# Autodesk Inventor assembly: prototype_5_batteryWithSlider
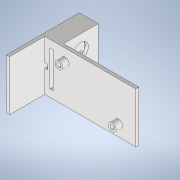
[picture p0: Inventor's stored thumbnail of the model, 180x180]
Saved by Autodesk Inventor 2022 (Build 260153000, 153)
## iProperties
Created: 2022-06-08
Part Number: prototype_5_batteryWithSlider
Document SubType Name: Assembly
Designer: tecware
Author: tecware
## Documents named in this file (3)
- C:\Users\tecware\Documents\git\calibrationKit\calibrationKit_v2\wand\prototype\New folder\prototype_6_batteryWithSlider.iam
- C:\Users\tecware\Documents\git\calibrationKit\calibrationKit_v2\wand\prototype\New folder\prototype_6_batteryPart.ipt
- C:\Users\tecware\Documents\git\calibrationKit\calibrationKit_v2\wand\prototype\New folder\prototype_6_sliderPart.ipt
## Components (2 placed, 2 different names)
1. prototype_6_batteryPart:1 — Mate:1, Mate:2
2. prototype_6_sliderPart:1 — Mate:1, Mate:2
## Relationships (2: Mate 2)
- Mate:1 (0.2 mm): prototype_6_batteryPart:1 ↔ prototype_6_sliderPart:1
- Mate:2 (0.2 mm): prototype_6_batteryPart:1 ↔ prototype_6_sliderPart:1
